# Autodesk Inventor assembly: tri-slot-feedlines
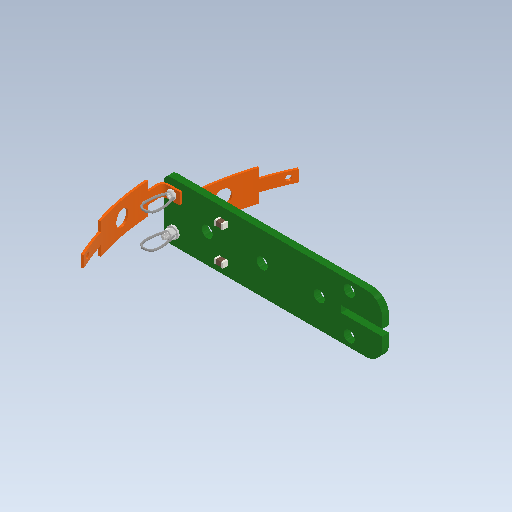
[picture p0: Inventor's stored thumbnail of the model, 512x512]
Saved by Autodesk Inventor 2021 (Build 250183000, 183)
## iProperties
Company: A Company
Created: 2020-02-27
Part Number: tri-slot-feedlines
Description: KiCad electronic assembly
Document SubType Name: Assembly
Designer: dsouthall
Authority: Unknown
Sending System: KiCad to STEP converter
Preprocessor: Open CASCADE STEP processor 6.9
Title: tri-slot-feedlines.step
Author: An Author
## Documents named in this file (8)
- C:\Users\dsouthall\OneDrive - The University of Chicago\Hpol\Model\source\feedlines\tri-slot-feedlines.iam
- C:\Users\dsouthall\OneDrive - The University of Chicago\Hpol\Model\source\feedlines\C_0805_2012Metric.iam
- C:\Users\dsouthall\OneDrive - The University of Chicago\Hpol\Model\source\feedlines\TestPoint_Loop_D3.80mm_Drill2.0mm.iam
- C:\Users\dsouthall\OneDrive - The University of Chicago\Hpol\Model\source\feedlines\COMPOUND.ipt
- C:\Users\dsouthall\OneDrive - The University of Chicago\Hpol\Model\source\digikey-mockup-A114140-ND.ipt
- C:\Users\dsouthall\OneDrive - The University of Chicago\Hpol\Model\source\92141A207_TYPE 18-8 STAINLESS STEEL FLAT WASHER\92141A207_TYPE 18-8 STAINLESS STEEL FLAT WASHER.ipt
- C:\Users\dsouthall\OneDrive - The University of Chicago\Hpol\Model\source\90001A403_TYPE 18-8 STAINLESS STEEL HEX NUT\90001A403_TYPE 18-8 STAINLESS STEEL HEX NUT.ipt
- C:\Users\dsouthall\OneDrive - The University of Chicago\Hpol\Model\source\90910A632_LOW-PROFILE BUTTON HEAD TORX MACHINE SCREW\90910A632_LOW-PROFILE BUTTON HEAD TORX MACHINE SCREW.ipt
## Components (13 placed, 9 different names)
1. 2 [sub-assembly] — Flush:2, Mate:1, Flush:3
2. 3 [sub-assembly] — Flush:1, Mate:2, Flush:4
3. 5 [sub-assembly]
4. 6 [sub-assembly]
5. 7 — Flush:1, Flush:2, Mate:1, Mate:2, Flush:3, Flush:4, Mate:3, Mate:4, Angle:1, Mate:5, Mate:6, Angle:2, Insert:5, Insert:6
6. digikey-mockup-A114140-ND:1 — Mate:3, Mate:4, Angle:1, Insert:11
7. digikey-mockup-A114140-ND:2 — Mate:5, Mate:6, Angle:2, Insert:12
8. 92141A207_TYPE 18-8 STAINLESS STEEL FLAT WASHER:1 — Insert:5, Insert:9
9. 92141A207_TYPE 18-8 STAINLESS STEEL FLAT WASHER:2 — Insert:6, Insert:10
10. 90001A403_TYPE 18-8 STAINLESS STEEL HEX NUT:1 — Insert:10
11. 90001A403_TYPE 18-8 STAINLESS STEEL HEX NUT:2 — Insert:9
12. 90910A632_LOW-PROFILE BUTTON HEAD TORX MACHINE SCREW:1 — Insert:11
13. 90910A632_LOW-PROFILE BUTTON HEAD TORX MACHINE SCREW:2 — Insert:12
## Relationships (18: Mate 6, Insert 6, Flush 4, Angle 2)
- Flush:1 (13.5 mm): 3 ↔ 7
- Flush:2 (13.5 mm): 2 ↔ 7
- Mate:1: 2 ↔ 7
- Mate:2: 3 ↔ 7
- Flush:3 (2.375 mm): 2 ↔ 7
- Flush:4 (2.375 mm): 3 ↔ 7
- Mate:3: 7 ↔ digikey-mockup-A114140-ND:1
- Mate:4: 7 ↔ digikey-mockup-A114140-ND:1
- Angle:1 (90 deg): 7 ↔ digikey-mockup-A114140-ND:1
- Mate:5: 7 ↔ digikey-mockup-A114140-ND:2
- Mate:6: 7 ↔ digikey-mockup-A114140-ND:2
- Angle:2 (180 deg): 7 ↔ digikey-mockup-A114140-ND:2
- Insert:5: 7 ↔ 92141A207_TYPE 18-8 STAINLESS STEEL FLAT WASHER:1
- Insert:6: 7 ↔ 92141A207_TYPE 18-8 STAINLESS STEEL FLAT WASHER:2
- Insert:9: 92141A207_TYPE 18-8 STAINLESS STEEL FLAT WASHER:1 ↔ 90001A403_TYPE 18-8 STAINLESS STEEL HEX NUT:2
- Insert:10: 92141A207_TYPE 18-8 STAINLESS STEEL FLAT WASHER:2 ↔ 90001A403_TYPE 18-8 STAINLESS STEEL HEX NUT:1
- Insert:11: digikey-mockup-A114140-ND:1 ↔ 90910A632_LOW-PROFILE BUTTON HEAD TORX MACHINE SCREW:1
- Insert:12: digikey-mockup-A114140-ND:2 ↔ 90910A632_LOW-PROFILE BUTTON HEAD TORX MACHINE SCREW:2
